# Autodesk Inventor assembly: assembled_v2
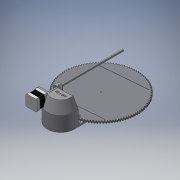
[picture p0: Inventor's stored thumbnail of the model, 180x180]
Saved by Autodesk Inventor 2016 (Build 200138000, 138)
## iProperties
Created: 2016-10-03
Part Number: assembled_v2
Document SubType Name: Assembly
Designer: brent
Author: brent
## Documents named in this file (4)
- C:\Users\brent\OneDrive\classes\desinv22\motorized_drawing_machine\assembled_v2.iam
- C:\Users\brent\OneDrive\classes\desinv22\motorized_drawing_machine\offtheshelf\nema17_40mm_300mml.ipt
- C:\Users\brent\OneDrive\classes\desinv22\motorized_drawing_machine\offtheshelf\nema17_33mm.ipt
- C:\Users\brent\OneDrive\classes\desinv22\motorized_drawing_machine\primary_v2.ipt
## Components (3 placed, 3 different names)
1. nema17_40mm_300mml:1 — Mate:2, Mate:5
2. nema17_33mm:1 — Mate:3, Mate:4
3. primary_v2:1 — Mate:1, Mate:2, Mate:3, Mate:4, Mate:5
## Relationships (5: Mate 5)
- Mate:1: primary_v2:1
- Mate:2: nema17_40mm_300mml:1 ↔ primary_v2:1
- Mate:3: nema17_33mm:1 ↔ primary_v2:1
- Mate:4: nema17_33mm:1 ↔ primary_v2:1
- Mate:5: nema17_40mm_300mml:1 ↔ primary_v2:1
